# Autodesk Inventor assembly: Thrust_Bench_Ball
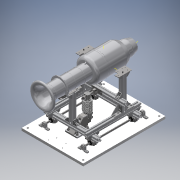
[picture p0: Inventor's stored thumbnail of the model, 180x180]
Saved by Autodesk Inventor 2019 (Build 230136000, 136)
## iProperties
Created: 2021-03-14
Part Number: Thrust_Bench_Ball
Document SubType Name: Assembly
Designer: rtavi
Author: rtavi
## Documents named in this file (19)
- C:\Users\rtavi\Desktop\GitHub\Micro-Turbojet_Test-Rig\StructureDesign\Thrust_Bench.iam
- C:\Users\rtavi\Desktop\GitHub\Micro-Turbojet_Test-Rig\StructureDesign\DesignedParts\Base.ipt
- C:\Users\rtavi\Desktop\GitHub\Micro-Turbojet_Test-Rig\StructureDesign\CommercialParts\Support_LSCS8.ipt
- C:\Users\rtavi\Desktop\GitHub\Micro-Turbojet_Test-Rig\StructureDesign\CommercialParts\Shaft_LJMR8.ipt
- C:\Users\rtavi\Desktop\GitHub\Micro-Turbojet_Test-Rig\StructureDesign\CommercialParts\Bearing_LUCS8.ipt
- C:\Users\rtavi\Desktop\GitHub\Micro-Turbojet_Test-Rig\StructureDesign\CommercialParts\Horizontal_profile_260mm.ipt
- C:\Users\rtavi\Desktop\GitHub\Micro-Turbojet_Test-Rig\StructureDesign\CommercialParts\Bracket.ipt
- C:\Users\rtavi\Desktop\GitHub\Micro-Turbojet_Test-Rig\StructureDesign\CommercialParts\Vertical_profile_160mm.ipt
- C:\Users\rtavi\Desktop\GitHub\Micro-Turbojet_Test-Rig\StructureDesign\DesignedParts\Engine_Mounting.ipt
- C:\Users\rtavi\Desktop\GitHub\Micro-Turbojet_Test-Rig\StructureDesign\CommercialParts\Engine.ipt
- C:\Users\rtavi\Desktop\GitHub\Micro-Turbojet_Test-Rig\StructureDesign\CommercialParts\Engine_data.ipt
- C:\Users\rtavi\Desktop\GitHub\Micro-Turbojet_Test-Rig\StructureDesign\CommercialParts\Bracket_20X40.ipt
- C:\Users\rtavi\Desktop\GitHub\Micro-Turbojet_Test-Rig\StructureDesign\CommercialParts\Screws\m8-washer.ipt
- C:\Users\rtavi\Desktop\GitHub\Micro-Turbojet_Test-Rig\StructureDesign\CommercialParts\Spring_751556.ipt
- C:\Users\rtavi\Desktop\GitHub\Micro-Turbojet_Test-Rig\StructureDesign\DesignedParts\Mounting_Shaft.ipt
- C:\Users\rtavi\Desktop\GitHub\Micro-Turbojet_Test-Rig\StructureDesign\Thrust_Measure.iam
- C:\Users\rtavi\Desktop\GitHub\Micro-Turbojet_Test-Rig\StructureDesign\Bellmouth\Bellmouth.ipt
- C:\Users\rtavi\Desktop\GitHub\Micro-Turbojet_Test-Rig\StructureDesign\Bellmouth\Bellmouth_union.ipt
- C:\Users\rtavi\Desktop\GitHub\Micro-Turbojet_Test-Rig\StructureDesign\CommercialParts\Vertical_profile_127mm.ipt
## Components (60 placed, 18 different names)
1. Base:1 — Flush:1, Flush:2, Flush:3, Mate:1, Mate:2, Mate:3, Mate:4, Mate:162
2. Engine:1 — Mate:187, Flush:133, Flush:134, Flush:135, Mate:188, Mate:189, Flush:191
3. Engine_data:1 — Mate:187
4. Thrust_Measure:1 [sub-assembly] — Flush:130, Mate:162, Mate:163, Flush:131
5. Support_LSCS8:1 — Mate:1, Insert:1
6. Support_LSCS8:2 — Mate:2, Insert:4
7. Support_LSCS8:3 — Mate:3, Insert:2, Mate:152, Mate:158
8. Support_LSCS8:4 — Mate:4, Insert:3, Mate:156
9. Shaft_LJMR8:1 — Mate:5, Insert:1, Insert:2, Mate:9, Mate:10, Mate:16, Mate:149, Mate:151, Mate:157, Mate:175
10. Shaft_LJMR8:2 — Mate:6, Insert:3, Insert:4, Mate:7, Mate:8, Mate:15, Mate:104, Mate:105, Mate:153, Mate:155, Mate:159, Mate:177
11. Bearing_LUCS8:1 — Mate:7, Mate:11, Flush:5, Mate:154
12. Bearing_LUCS8:2 — Mate:8, Mate:13, Flush:7
13. Bearing_LUCS8:3 — Mate:9, Mate:12, Flush:4, Mate:150, Mate:158
14. Bearing_LUCS8:4 — Mate:10, Mate:14, Flush:6
15. m8-washer:1 — Mate:149, Mate:150, Mate:174
16. m8-washer:2 — Mate:151, Mate:152
17. m8-washer:3 — Mate:153, Mate:154, Mate:176
18. m8-washer:4 — Mate:155, Mate:156
19. m8-washer:5 — Mate:174, Mate:175
20. m8-washer:6 — Mate:176, Mate:177
21. Spring_751556:1 — Mate:157
22. Spring_751556:2 — Mate:159
23. Horizontal_profile_260mm:1 — Mate:11, Mate:12, Flush:4, Flush:5, Mate:21, Mate:22, Mate:24, Mate:29, Mate:35, Mate:41, Mate:47, Mate:105, Flush:125
24. Horizontal_profile_260mm:2 — Mate:13, Mate:14, Flush:6, Flush:7, Mate:21, Mate:23, Mate:25, Mate:26, Mate:32, Mate:39, Mate:44, Flush:15, Mate:104, Flush:118, Mate:192, Flush:136, Mate:193, Mate:195
25. Horizontal_profile_260mm:3 — Mate:22, Mate:23, Mate:27, Mate:28, Mate:30, Mate:31, Mate:33, Mate:34, Mate:36, Mate:37, Mate:50, Flush:14, Flush:117, Flush:125, Mate:144, Mate:145
26. Horizontal_profile_260mm:4 — Mate:24, Mate:25, Mate:38, Mate:40, Mate:42, Mate:43, Mate:45, Mate:46, Mate:48, Mate:49, Mate:51, Flush:13, Flush:116, Mate:139, Mate:141
27. Bracket:1 — Mate:26, Mate:27, Mate:28, Flush:117
28. Bracket:2 — Mate:29, Mate:30, Mate:31
29. Bracket:3 — Mate:32, Mate:33, Mate:34
30. Bracket:4 — Mate:35, Mate:36, Mate:37
31. Bracket:5 — Mate:38, Mate:39, Mate:40, Flush:116
32. Bracket:6 — Mate:41, Mate:42, Mate:43
33. Bracket:7 — Mate:44, Mate:45, Mate:46
34. Bracket:8 — Mate:47, Mate:48, Mate:49
35. Vertical_profile_160mm:1 — Mate:50, Flush:14, Mate:52, Flush:118, Mate:126, Mate:131, Mate:128, Mate:129, Flush:122, Mate:133, Mate:135, Mate:138, Mate:143, Mate:146, Mate:147, Mate:148, Mate:161, Flush:129, Mate:165, Mate:184, Mate:186, Flush:135
36. Vertical_profile_160mm:2 — Mate:51, Flush:13, Mate:53, Mate:93, Mate:121, Flush:121, Mate:123, Mate:125, Flush:123, Mate:132, Mate:134, Mate:137, Mate:140, Mate:142, Flush:126, Flush:127, Mate:160, Flush:128, Mate:172, Mate:182, Mate:183
37. Horizontal_profile_260mm:5 — Mate:52, Mate:53, Flush:15, Mate:163, Flush:131, Mate:164, Flush:132, Mate:171, Mate:173, Mate:181, Mate:185
38. Bracket:9 — Mate:164, Mate:165, Flush:132
39. Bracket:10 — Mate:184, Mate:185, Mate:186
40. Bracket:11 — Mate:171, Mate:172, Mate:173
41. Bracket:12 — Mate:181, Mate:182, Mate:183
42. Bracket_20X40:1 — Mate:139, Mate:140, Flush:126
43. Bracket_20X40:2 — Mate:141, Mate:142, Flush:127
44. Bracket_20X40:3 — Mate:143, Mate:144, Mate:147
45. Bracket_20X40:4 — Mate:145, Mate:146, Mate:148
46. Engine_Mounting:1 — Mate:93, Mate:100, Symmetry:1, Symmetry:2, Mate:127, Mate:130, Flush:122, Flush:124, Mate:133, Mate:135, Mate:138
47. Engine_Mounting:2 — Mate:100, Symmetry:1, Symmetry:2, Mate:122, Mate:124, Flush:123, Flush:124, Mate:132, Mate:134, Mate:137, Flush:134
48. Bracket:13 — Mate:121, Mate:122, Flush:121
49. Bracket:14 — Mate:123, Mate:124, Mate:125
50. Bracket:15 — Mate:131, Mate:129, Mate:130
51. Bracket:16 — Mate:126, Mate:127, Mate:128
52. Mounting_Shaft:1 — Mate:161, Flush:129
53. Mounting_Shaft:2 — Mate:160, Flush:128
54. Bellmouth:1 — Mate:188, Mate:189, Flush:191, Mate:191, Tangent:1, Tangent:2, Tangent:3
55. Bellmouth_union:1 — Mate:191, Tangent:1, Tangent:2, Tangent:3
56. Vertical_profile_127mm:1 — Mate:192, Flush:136, Flush:137, Mate:194, Mate:196, Mate:197, Flush:138, Mate:198, Flush:139, Mate:199, Flush:140, Flush:141, Mate:200
57. Bracket:17 — Mate:193, Mate:194, Mate:197
58. Bracket:18 — Mate:195, Mate:196, Flush:138
59. Bracket:19 — Mate:198, Flush:139, Flush:141
60. Bracket:20 — Mate:199, Flush:140, Mate:200
## Relationships (167: Mate 123, Flush 35, Insert 4, Tangent 3, Symmetry 2)
- Flush:1: Base:1
- Flush:2: Base:1
- Flush:3: Base:1
- Mate:1: Base:1 ↔ Support_LSCS8:1
- Mate:2: Base:1 ↔ Support_LSCS8:2
- Mate:3: Base:1 ↔ Support_LSCS8:3
- Mate:4: Base:1 ↔ Support_LSCS8:4
- Mate:5: Shaft_LJMR8:1
- Mate:6: Shaft_LJMR8:2
- Insert:1 (0.2 mm): Support_LSCS8:1 ↔ Shaft_LJMR8:1
- Insert:2 (0.2 mm): Support_LSCS8:3 ↔ Shaft_LJMR8:1
- Insert:3 (0.2 mm): Support_LSCS8:4 ↔ Shaft_LJMR8:2
- Insert:4 (-0.2 mm): Support_LSCS8:2 ↔ Shaft_LJMR8:2
- Mate:7: Shaft_LJMR8:2 ↔ Bearing_LUCS8:1
- Mate:8: Shaft_LJMR8:2 ↔ Bearing_LUCS8:2
- Mate:9: Shaft_LJMR8:1 ↔ Bearing_LUCS8:3
- Mate:10: Shaft_LJMR8:1 ↔ Bearing_LUCS8:4
- Mate:11: Bearing_LUCS8:1 ↔ Horizontal_profile_260mm:1
- Mate:12: Bearing_LUCS8:3 ↔ Horizontal_profile_260mm:1
- Mate:13: Bearing_LUCS8:2 ↔ Horizontal_profile_260mm:2
- Mate:14: Bearing_LUCS8:4 ↔ Horizontal_profile_260mm:2
- Flush:4 (3.7 mm): Bearing_LUCS8:3 ↔ Horizontal_profile_260mm:1
- Flush:5 (3.7 mm): Bearing_LUCS8:1 ↔ Horizontal_profile_260mm:1
- Flush:6 (3.7 mm): Bearing_LUCS8:4 ↔ Horizontal_profile_260mm:2
- Flush:7 (3.7 mm): Bearing_LUCS8:2 ↔ Horizontal_profile_260mm:2
- Mate:15 (-95 mm): Shaft_LJMR8:2
- Mate:16 (95 mm): Shaft_LJMR8:1
- Mate:21 (180 mm): Horizontal_profile_260mm:1 ↔ Horizontal_profile_260mm:2
- Mate:22: Horizontal_profile_260mm:1 ↔ Horizontal_profile_260mm:3
- Mate:23: Horizontal_profile_260mm:2 ↔ Horizontal_profile_260mm:3
- Mate:24: Horizontal_profile_260mm:1 ↔ Horizontal_profile_260mm:4
- Mate:25: Horizontal_profile_260mm:2 ↔ Horizontal_profile_260mm:4
- Mate:26: Horizontal_profile_260mm:2 ↔ Bracket:1
- Mate:27: Horizontal_profile_260mm:3 ↔ Bracket:1
- Mate:28: Horizontal_profile_260mm:3 ↔ Bracket:1
- Mate:29: Horizontal_profile_260mm:1 ↔ Bracket:2
- Mate:30: Horizontal_profile_260mm:3 ↔ Bracket:2
- Mate:31: Horizontal_profile_260mm:3 ↔ Bracket:2
- Mate:32: Horizontal_profile_260mm:2 ↔ Bracket:3
- Mate:33: Horizontal_profile_260mm:3 ↔ Bracket:3
- Mate:34: Horizontal_profile_260mm:3 ↔ Bracket:3
- Mate:35: Horizontal_profile_260mm:1 ↔ Bracket:4
- Mate:36: Horizontal_profile_260mm:3 ↔ Bracket:4
- Mate:37: Horizontal_profile_260mm:3 ↔ Bracket:4
- Mate:38: Horizontal_profile_260mm:4 ↔ Bracket:5
- Mate:39: Horizontal_profile_260mm:2 ↔ Bracket:5
- Mate:40: Horizontal_profile_260mm:4 ↔ Bracket:5
- Mate:41: Horizontal_profile_260mm:1 ↔ Bracket:6
- Mate:42: Horizontal_profile_260mm:4 ↔ Bracket:6
- Mate:43: Horizontal_profile_260mm:4 ↔ Bracket:6
- Mate:44: Horizontal_profile_260mm:2 ↔ Bracket:7
- Mate:45: Horizontal_profile_260mm:4 ↔ Bracket:7
- Mate:46: Horizontal_profile_260mm:4 ↔ Bracket:7
- Mate:47: Horizontal_profile_260mm:1 ↔ Bracket:8
- Mate:48: Horizontal_profile_260mm:4 ↔ Bracket:8
- Mate:49: Horizontal_profile_260mm:4 ↔ Bracket:8
- Mate:50: Horizontal_profile_260mm:3 ↔ Vertical_profile_160mm:1
- Mate:51: Horizontal_profile_260mm:4 ↔ Vertical_profile_160mm:2
- Flush:13: Horizontal_profile_260mm:4 ↔ Vertical_profile_160mm:2
- Flush:14: Horizontal_profile_260mm:3 ↔ Vertical_profile_160mm:1
- Mate:52: Vertical_profile_160mm:1 ↔ Horizontal_profile_260mm:5
- Mate:53: Vertical_profile_160mm:2 ↔ Horizontal_profile_260mm:5
- Flush:15: Horizontal_profile_260mm:2 ↔ Horizontal_profile_260mm:5
- Mate:93: Vertical_profile_160mm:2 ↔ Engine_Mounting:1
- Mate:100 (156 mm): Engine_Mounting:1 ↔ Engine_Mounting:2
- Symmetry:1: Engine_Mounting:1 ↔ Engine_Mounting:2
- Symmetry:2: Engine_Mounting:1 ↔ Engine_Mounting:2
- Mate:104 (-35 mm): Shaft_LJMR8:2 ↔ Horizontal_profile_260mm:2
- Mate:105 (-35 mm): Shaft_LJMR8:2 ↔ Horizontal_profile_260mm:1
- Flush:116 (-2 mm): Horizontal_profile_260mm:4 ↔ Bracket:5
- Flush:117 (-2 mm): Horizontal_profile_260mm:3 ↔ Bracket:1
- Flush:118 (-150 mm): Horizontal_profile_260mm:2 ↔ Vertical_profile_160mm:1
- Mate:121: Vertical_profile_160mm:2 ↔ Bracket:13
- Mate:122: Engine_Mounting:2 ↔ Bracket:13
- Flush:121: Vertical_profile_160mm:2 ↔ Bracket:13
- Mate:123: Vertical_profile_160mm:2 ↔ Bracket:14
- Mate:124: Engine_Mounting:2 ↔ Bracket:14
- Mate:125: Vertical_profile_160mm:2 ↔ Bracket:14
- Mate:126: Vertical_profile_160mm:1 ↔ Bracket:16
- Mate:127: Engine_Mounting:1 ↔ Bracket:16
- Mate:131: Vertical_profile_160mm:1 ↔ Bracket:15
- Mate:128: Vertical_profile_160mm:1 ↔ Bracket:16
- Mate:129: Vertical_profile_160mm:1 ↔ Bracket:15
- Mate:130: Engine_Mounting:1 ↔ Bracket:15
- Flush:122: Vertical_profile_160mm:1 ↔ Engine_Mounting:1
- Flush:123: Vertical_profile_160mm:2 ↔ Engine_Mounting:2
- Flush:124: Engine_Mounting:1 ↔ Engine_Mounting:2
- Mate:132: Vertical_profile_160mm:2 ↔ Engine_Mounting:2
- Mate:133: Vertical_profile_160mm:1 ↔ Engine_Mounting:1
- Mate:134: Vertical_profile_160mm:2 ↔ Engine_Mounting:2
- Mate:135: Vertical_profile_160mm:1 ↔ Engine_Mounting:1
- Mate:137: Vertical_profile_160mm:2 ↔ Engine_Mounting:2
- Mate:138: Vertical_profile_160mm:1 ↔ Engine_Mounting:1
- Flush:125 (-25 mm): Horizontal_profile_260mm:1 ↔ Horizontal_profile_260mm:3
- Mate:139: Horizontal_profile_260mm:4 ↔ Bracket_20X40:1
- Mate:140: Vertical_profile_160mm:2 ↔ Bracket_20X40:1
- Mate:141: Horizontal_profile_260mm:4 ↔ Bracket_20X40:2
- Mate:142: Vertical_profile_160mm:2 ↔ Bracket_20X40:2
- Flush:126: Vertical_profile_160mm:2 ↔ Bracket_20X40:1
- Flush:127: Vertical_profile_160mm:2 ↔ Bracket_20X40:2
- Mate:143: Vertical_profile_160mm:1 ↔ Bracket_20X40:3
- Mate:144: Horizontal_profile_260mm:3 ↔ Bracket_20X40:3
- Mate:145: Horizontal_profile_260mm:3 ↔ Bracket_20X40:4
- Mate:146: Vertical_profile_160mm:1 ↔ Bracket_20X40:4
- Mate:147: Vertical_profile_160mm:1 ↔ Bracket_20X40:3
- Mate:148: Vertical_profile_160mm:1 ↔ Bracket_20X40:4
- Mate:149: Shaft_LJMR8:1 ↔ m8-washer:1
- Mate:150: Bearing_LUCS8:3 ↔ m8-washer:1
- Mate:151: Shaft_LJMR8:1 ↔ m8-washer:2
- Mate:152: Support_LSCS8:3 ↔ m8-washer:2
- Mate:153: Shaft_LJMR8:2 ↔ m8-washer:3
- Mate:154: Bearing_LUCS8:1 ↔ m8-washer:3
- Mate:155: Shaft_LJMR8:2 ↔ m8-washer:4
- Mate:156: Support_LSCS8:4 ↔ m8-washer:4
- Mate:157: Shaft_LJMR8:1 ↔ Spring_751556:1
- Mate:158 (29.2 mm): Support_LSCS8:3 ↔ Bearing_LUCS8:3
- Mate:159: Shaft_LJMR8:2 ↔ Spring_751556:2
- Mate:160: Vertical_profile_160mm:2 ↔ Mounting_Shaft:2
- Flush:128: Vertical_profile_160mm:2 ↔ Mounting_Shaft:2
- Mate:161: Vertical_profile_160mm:1 ↔ Mounting_Shaft:1
- Flush:129: Vertical_profile_160mm:1 ↔ Mounting_Shaft:1
- Flush:130: Thrust_Measure:1
- Mate:162: Base:1 ↔ Thrust_Measure:1
- Mate:163: Thrust_Measure:1 ↔ Horizontal_profile_260mm:5
- Flush:131: Thrust_Measure:1 ↔ Horizontal_profile_260mm:5
- Mate:164: Horizontal_profile_260mm:5 ↔ Bracket:9
- Mate:165: Vertical_profile_160mm:1 ↔ Bracket:9
- Flush:132: Horizontal_profile_260mm:5 ↔ Bracket:9
- Mate:171: Horizontal_profile_260mm:5 ↔ Bracket:11
- Mate:172: Vertical_profile_160mm:2 ↔ Bracket:11
- Mate:173: Horizontal_profile_260mm:5 ↔ Bracket:11
- Mate:174: m8-washer:1 ↔ m8-washer:5
- Mate:175: Shaft_LJMR8:1 ↔ m8-washer:5
- Mate:176: m8-washer:3 ↔ m8-washer:6
- Mate:177: Shaft_LJMR8:2 ↔ m8-washer:6
- Mate:181: Horizontal_profile_260mm:5 ↔ Bracket:12
- Mate:182: Vertical_profile_160mm:2 ↔ Bracket:12
- Mate:183: Vertical_profile_160mm:2 ↔ Bracket:12
- Mate:184: Vertical_profile_160mm:1 ↔ Bracket:10
- Mate:185: Horizontal_profile_260mm:5 ↔ Bracket:10
- Mate:186: Vertical_profile_160mm:1 ↔ Bracket:10
- Mate:187: Engine:1 ↔ Engine_data:1
- Flush:133: Engine:1
- Flush:134: Engine:1 ↔ Engine_Mounting:2
- Flush:135: Engine:1 ↔ Vertical_profile_160mm:1
- Mate:188: Engine:1 ↔ Bellmouth:1
- Mate:189: Engine:1 ↔ Bellmouth:1
- Flush:191: Engine:1 ↔ Bellmouth:1
- Mate:191: Bellmouth:1 ↔ Bellmouth_union:1
- Tangent:1: Bellmouth:1 ↔ Bellmouth_union:1
- Tangent:2: Bellmouth:1 ↔ Bellmouth_union:1
- Tangent:3: Bellmouth:1 ↔ Bellmouth_union:1
- Mate:192: Horizontal_profile_260mm:2 ↔ Vertical_profile_127mm:1
- Flush:136: Horizontal_profile_260mm:2 ↔ Vertical_profile_127mm:1
- Flush:137: Vertical_profile_127mm:1
- Mate:193: Horizontal_profile_260mm:2 ↔ Bracket:17
- Mate:194: Vertical_profile_127mm:1 ↔ Bracket:17
- Mate:195: Horizontal_profile_260mm:2 ↔ Bracket:18
- Mate:196: Vertical_profile_127mm:1 ↔ Bracket:18
- Mate:197: Vertical_profile_127mm:1 ↔ Bracket:17
- Flush:138: Vertical_profile_127mm:1 ↔ Bracket:18
- Mate:198: Vertical_profile_127mm:1 ↔ Bracket:19
- Flush:139: Vertical_profile_127mm:1 ↔ Bracket:19
- Mate:199: Vertical_profile_127mm:1 ↔ Bracket:20
- Flush:140: Vertical_profile_127mm:1 ↔ Bracket:20
- Flush:141: Vertical_profile_127mm:1 ↔ Bracket:19
- Mate:200: Vertical_profile_127mm:1 ↔ Bracket:20
## Named parameters: sa_0 = -1.2e-12, sa_1 = -0, sa_2 = -1667.7, sa_3 = 981, sa_4 = 20000
note: some values were not read from the file. Shown as the stored number, unit unknown: "sa_0", "sa_1", "sa_2", "sa_3", "sa_4".
